# Autodesk Inventor assembly: ASM Heating Unit
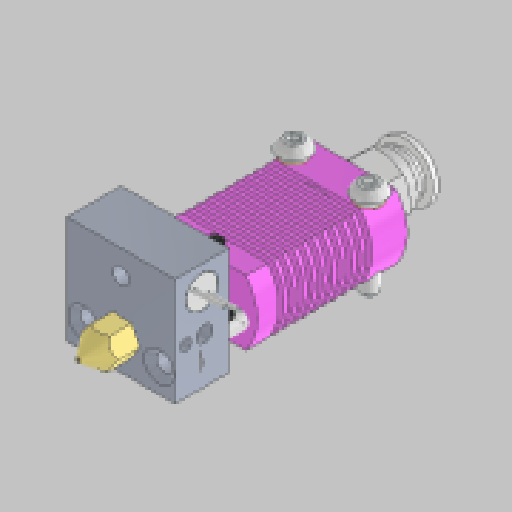
[picture p0: Inventor's stored thumbnail of the model, 512x512]
Saved by Autodesk Inventor 2025.3 (Build 293356000, 356)
## iProperties
Created: 2022-04-13
Part Number: ASM Heating Unit
Document SubType Name: Assembly
Designer: javie
Author: javie
Revision Number: ANY
## Documents named in this file (11)
- C:\Users\Inema\OneDrive - INEMA S.A\Escritorio\Modelo Ender 3\ASM Heating Unit.iam
- C:\Users\Inema\OneDrive - INEMA S.A\Escritorio\Modelo Ender 3\Radiator.ipt
- C:\Users\Inema\OneDrive - INEMA S.A\Escritorio\Modelo Ender 3\nozzle.ipt
- C:\Users\Inema\OneDrive - INEMA S.A\Escritorio\Modelo Ender 3\Heat block.ipt
- C:\Users\Inema\OneDrive - INEMA S.A\Escritorio\Modelo Ender 3\Pneumatic joint.ipt
- C:\Users\Inema\OneDrive - INEMA S.A\Escritorio\Modelo Ender 3\Nozzle thermistor.ipt
- C:\Users\Inema\OneDrive - INEMA S.A\Escritorio\Modelo Ender 3\Heater.ipt
- C:\Users\Inema\OneDrive - INEMA S.A\Escritorio\Modelo Ender 3\M3X16 Pan Head Screw.ipt
- C:\Users\Inema\OneDrive - INEMA S.A\Escritorio\Modelo Ender 3\M3 Split Washer.ipt
- C:\Users\Inema\OneDrive - INEMA S.A\Escritorio\Modelo Ender 3\M3×18 Flush Head Screw.ipt
- C:\Users\Inema\OneDrive - INEMA S.A\Escritorio\Modelo Ender 3\M3 Screw.ipt
## Components (14 placed, 14 different names)
1. Radiator_200 — Coincidencia:3
2. nozzle_201 — Insertar:1, Coincidencia:3
3. Heat block_202 — Insertar:1, Insertar:2, Coincidencia:1, Coincidencia:2
4. Pneumatic joint_203
5. Nozzle thermistor_204
6. Heater_205 — Insertar:2
7. M3X16 Pan Head Screw_206
8. M3 Split Washer_207
9. M3×18 Flush Head Screw_208 — Coincidencia:1
10. M3×18 Flush Head Screw_209 — Coincidencia:2
11. M3 Screw_210
12. M3X16 Pan Head Screw_211
13. M3 Split Washer_212
14. M3 Screw_213
## Relationships (5: Mate 3, Insert 2)
- Insertar:1: nozzle_201 ↔ Heat block_202
- Insertar:2: Heat block_202 ↔ Heater_205
- Coincidencia:1 [Mate]: Heat block_202 ↔ M3×18 Flush Head Screw_208
- Coincidencia:2 [Mate]: Heat block_202 ↔ M3×18 Flush Head Screw_209
- Coincidencia:3 [Mate] (-51 mm): Radiator_200 ↔ nozzle_201
